# Autodesk Inventor assembly: 810004_Power Shield ASSY
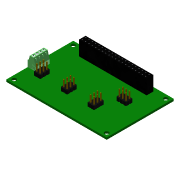
[picture p0: Inventor's stored thumbnail of the model, 180x180]
Saved by Autodesk Inventor 2015 (Build 190159000, 159)
## iProperties
Created: 2014-08-12
Part Number: 810004_Power Shield ASSY
Document SubType Name: Assembly
Designer: david
Author: david
## Documents named in this file (5)
- C:\SharedDrive\Dropbox\FAST Robotics\Products\818004_Power Shield\MECH\810004_Power Shield\810004A\810004A_XXX.iam
- C:\SharedDrive\Dropbox\FAST Robotics\Library\784006_Phoenix 4pos .1in\MECH\784006_Phoenix 4pos .1in.iam
- C:\SharedDrive\Dropbox\FAST Robotics\Library\784001_CONN HEADER .1in SINGLE STR 40POS\CONN HEADER .1in SINGLE STR 40POS.ipt
- C:\SharedDrive\Dropbox\FAST Robotics\Products\818004_Power Shield\MECH\818002_Power Shield Bare PCB\818002A\818002A_Power Shield Bare PCB.ipt
- C:\SharedDrive\Dropbox\FAST Robotics\Library\784009_PC104 Connector\784009_PC104 Connector.ipt
## Components (27 placed, 4 different names)
1. 818002A_Power Shield Bare PCB:1 — Flush:1, Flush:2, Flush:3, Mate:7, Flush:9, Flush:10, Mate:9, Mate:10, Mate:11, Mate:12, Mate:13, Flush:18, Mate:14
2. 784006_Phoenix 4pos .1in:1 [sub-assembly] — Mate:7, Flush:9, Flush:10
3. 784009_PC104 Connector:1 — Mate:13, Flush:18, Mate:14
4. CONN HEADER .1in SINGLE STR 40POS:7
5. CONN HEADER .1in SINGLE STR 40POS:8 — Mate:11
6. CONN HEADER .1in SINGLE STR 40POS:9
7. CONN HEADER .1in SINGLE STR 40POS:10
8. CONN HEADER .1in SINGLE STR 40POS:11 — Flush:17
9. CONN HEADER .1in SINGLE STR 40POS:12
10. CONN HEADER .1in SINGLE STR 40POS:13 — Flush:14
11. CONN HEADER .1in SINGLE STR 40POS:15 — Mate:10, Flush:17
12. CONN HEADER .1in SINGLE STR 40POS:16
13. CONN HEADER .1in SINGLE STR 40POS:17
14. CONN HEADER .1in SINGLE STR 40POS:18
15. CONN HEADER .1in SINGLE STR 40POS:19
16. CONN HEADER .1in SINGLE STR 40POS:14
17. CONN HEADER .1in SINGLE STR 40POS:20 — Mate:12
18. CONN HEADER .1in SINGLE STR 40POS:21
19. CONN HEADER .1in SINGLE STR 40POS:22
20. CONN HEADER .1in SINGLE STR 40POS:23
21. CONN HEADER .1in SINGLE STR 40POS:24
22. CONN HEADER .1in SINGLE STR 40POS:1
23. CONN HEADER .1in SINGLE STR 40POS:2 — Mate:9
24. CONN HEADER .1in SINGLE STR 40POS:3
25. CONN HEADER .1in SINGLE STR 40POS:4 — Flush:14
26. CONN HEADER .1in SINGLE STR 40POS:5
27. CONN HEADER .1in SINGLE STR 40POS:6
## Component patterns: (2 elements), (6 elements, first: CONN HEADER .1in SINGLE STR 40POS:7), (6 elements, first: CONN HEADER .1in SINGLE STR 40POS:13), (6 elements, first: CONN HEADER .1in SINGLE STR 40POS:14), (3 elements, first: CONN HEADER .1in SINGLE STR 40POS:1), Component Pattern 5:2 (3 elements)
## Relationships (15: Flush 8, Mate 7)
- Flush:1: 818002A_Power Shield Bare PCB:1
- Flush:2: 818002A_Power Shield Bare PCB:1
- Flush:3: 818002A_Power Shield Bare PCB:1
- Mate:7: 818002A_Power Shield Bare PCB:1 ↔ 784006_Phoenix 4pos .1in:1
- Flush:9: 818002A_Power Shield Bare PCB:1 ↔ 784006_Phoenix 4pos .1in:1
- Flush:10 (-24.13 mm): 818002A_Power Shield Bare PCB:1 ↔ 784006_Phoenix 4pos .1in:1
- Mate:9: 818002A_Power Shield Bare PCB:1 ↔ CONN HEADER .1in SINGLE STR 40POS:2
- Mate:10: 818002A_Power Shield Bare PCB:1 ↔ CONN HEADER .1in SINGLE STR 40POS:15
- Mate:11: 818002A_Power Shield Bare PCB:1 ↔ CONN HEADER .1in SINGLE STR 40POS:8
- Mate:12: 818002A_Power Shield Bare PCB:1 ↔ CONN HEADER .1in SINGLE STR 40POS:20
- Flush:14: CONN HEADER .1in SINGLE STR 40POS:13 ↔ CONN HEADER .1in SINGLE STR 40POS:4
- Flush:17: CONN HEADER .1in SINGLE STR 40POS:11 ↔ CONN HEADER .1in SINGLE STR 40POS:15
- Mate:13: 818002A_Power Shield Bare PCB:1 ↔ 784009_PC104 Connector:1
- Flush:18 (-4.318 mm): 818002A_Power Shield Bare PCB:1 ↔ 784009_PC104 Connector:1
- Mate:14 (-13.716 mm): 818002A_Power Shield Bare PCB:1 ↔ 784009_PC104 Connector:1
